# Autodesk Inventor assembly: Final Assembly
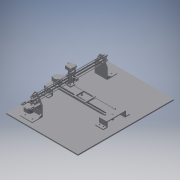
[picture p0: Inventor's stored thumbnail of the model, 180x180]
Saved by Autodesk Inventor 2019 (Build 230136000, 136)
## iProperties
Created: 2020-02-02
Document SubType Name: Assembly
Designer: Nishant
Author: Nishant
## Documents named in this file (20)
- D:\Desktop\College\Exploration\3d model\Final Assembly.iam
- D:\Desktop\College\Exploration\3d model\sheet.ipt
- D:\Desktop\College\Exploration\3d model\xaxis_clamp1.ipt
- D:\Desktop\College\Exploration\3d model\xaxis_clamp2.ipt
- D:\Desktop\College\Exploration\3d model\28byj48.ipt
- D:\Desktop\College\Exploration\3d model\gt2 16teeth pulley.ipt
- D:\Desktop\College\Exploration\3d model\pin.ipt
- D:\Desktop\College\Exploration\3d model\idler-pulley.ipt
- D:\Desktop\College\Exploration\3d model\belt1.ipt
- D:\Desktop\College\Exploration\3d model\xaxis_rod.ipt
- D:\Desktop\College\Exploration\3d model\zaxis_clamp2.ipt
- D:\Desktop\College\Exploration\3d model\zaxis_pin.ipt
- D:\Desktop\College\Exploration\3d model\zaxis_clamp1.ipt
- D:\Desktop\College\Exploration\3d model\yaxis_clamp2.ipt
- D:\Desktop\College\Exploration\3d model\yaxis_belt.ipt
- D:\Desktop\College\Exploration\3d model\yaxis_clamp1.ipt
- D:\Desktop\College\Exploration\3d model\yaxis_pin.ipt
- D:\Desktop\College\Exploration\3d model\yaxis_rod.ipt
- D:\Desktop\College\Exploration\3d model\yaxis_platform.ipt
- D:\Desktop\College\Exploration\3d model\SG90.ipt
## Components (25 placed, 19 different names)
1. sheet:1 — Rigid:1, Rigid:2, Rigid:10, Rotational:5
2. xaxis_clamp1:1 — Rigid:1, Rigid:3, Rotational:1, Rigid:8
3. xaxis_clamp2:1 — Rigid:2, Rigid:6
4. 28byj48:1 — Rigid:3, Rigid:4
5. gt2 16teeth pulley:1 — Rigid:4, Rigid:7
6. pin:1 — Rigid:5, Rigid:6
7. idler-pulley:1 — Rigid:5
8. belt1:1 — Rigid:7
9. xaxis_rod:1 — Rotational:1, Mate:1
10. xaxis_rod:2 — Rigid:8
11. zaxis_clamp2:1 — Mate:1, Rigid:9, Rotational:4, Rigid:17
12. zaxis_pin:1 — Rotational:2, Rigid:9
13. zaxis_pin:2 — Rotational:3, Rotational:4
14. zaxis_clamp1:1 — Rotational:2, Rotational:3
15. yaxis_clamp2:1 — Rigid:10, Rigid:11
16. 28byj48:2 — Rigid:11, Rigid:12
17. gt2 16teeth pulley:2 — Rigid:12, Rigid:13
18. yaxis_belt:1 — Rigid:13
19. yaxis_clamp1:1 — Rotational:5, Rigid:14, Rigid:15, Rigid:16
20. yaxis_pin:1 — Rigid:14, Rotational:6
21. idler-pulley:2 — Rotational:6
22. yaxis_rod:1 — Rigid:15
23. yaxis_rod:2 — Rigid:16
24. yaxis_platform:1
25. SG90:1 — Rigid:17
## Relationships (24: WeldJoint 17, RevoluteJoint 6, Mate 1)
- Rigid:1 [WeldJoint]: sheet:1 ↔ xaxis_clamp1:1
- Rigid:2 [WeldJoint]: sheet:1 ↔ xaxis_clamp2:1
- Rigid:3 [WeldJoint]: xaxis_clamp1:1 ↔ 28byj48:1
- Rigid:4 [WeldJoint] (-3 mm): 28byj48:1 ↔ gt2 16teeth pulley:1
- Rigid:5 [WeldJoint] (-6.75 mm): pin:1 ↔ idler-pulley:1
- Rigid:6 [WeldJoint]: xaxis_clamp2:1 ↔ pin:1
- Rigid:7 [WeldJoint] (0.5 mm): gt2 16teeth pulley:1 ↔ belt1:1
- Rotational:1 [RevoluteJoint] (-3.2 mm): xaxis_clamp1:1 ↔ xaxis_rod:1
- Rigid:8 [WeldJoint] (-3.2 mm): xaxis_clamp1:1 ↔ xaxis_rod:2
- Mate:1: xaxis_rod:1 ↔ zaxis_clamp2:1
- Rotational:2 [RevoluteJoint] (-14.5 mm): zaxis_pin:1 ↔ zaxis_clamp1:1
- Rotational:3 [RevoluteJoint] (-14.5 mm): zaxis_pin:2 ↔ zaxis_clamp1:1
- Rigid:9 [WeldJoint]: zaxis_clamp2:1 ↔ zaxis_pin:1
- Rotational:4 [RevoluteJoint]: zaxis_clamp2:1 ↔ zaxis_pin:2
- Rigid:10 [WeldJoint]: sheet:1 ↔ yaxis_clamp2:1
- Rigid:11 [WeldJoint]: yaxis_clamp2:1 ↔ 28byj48:2
- Rigid:12 [WeldJoint] (-3 mm): 28byj48:2 ↔ gt2 16teeth pulley:2
- Rigid:13 [WeldJoint] (-0.5 mm): gt2 16teeth pulley:2 ↔ yaxis_belt:1
- Rotational:5 [RevoluteJoint]: sheet:1 ↔ yaxis_clamp1:1
- Rigid:14 [WeldJoint]: yaxis_clamp1:1 ↔ yaxis_pin:1
- Rotational:6 [RevoluteJoint] (-1.5 mm): yaxis_pin:1 ↔ idler-pulley:2
- Rigid:15 [WeldJoint] (1 mm): yaxis_clamp1:1 ↔ yaxis_rod:1
- Rigid:16 [WeldJoint] (1 mm): yaxis_clamp1:1 ↔ yaxis_rod:2
- Rigid:17 [WeldJoint]: zaxis_clamp2:1 ↔ SG90:1
